# Autodesk Inventor assembly: Hand_tyokudou
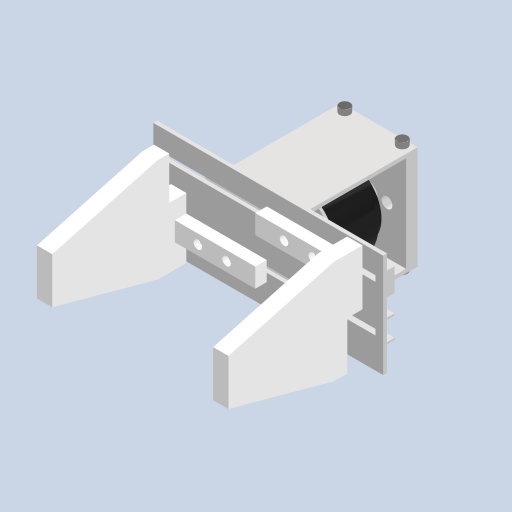
[picture p0: Inventor's stored thumbnail of the model, 512x512]
Saved by Autodesk Inventor 2023 (Build 270158000, 158)
## iProperties
Created: 2024-11-27
Part Number: Hand_tyokudou
Document SubType Name: Assembly
Designer: kiyo
Mass: 142.009 g
Surface Area: 718.919 cm^2
Volume: 132.865 cm^3
Density: 1.06882 g/cm^3
Author: kiyo
## Documents named in this file (14)
- D:\GitHub\inventor\syu-si\OfficeRobot\Manipulator\Hand_tyokudou.iam
- D:\GitHub\inventor\syu-si\OfficeRobot\ReadyMade\Steadywin\GIM3505-8_with-driver.ipt
- D:\GitHub\inventor\syu-si\OfficeRobot\Manipulator\rackgear.ipt
- D:\GitHub\inventor\syu-si\OfficeRobot\Manipulator\motor-fixing.ipt
- D:\GitHub\inventor\syu-si\OfficeRobot\Manipulator\hand-box.ipt
- D:\GitHub\inventor\syu-si\OfficeRobot\Manipulator\left-nail.ipt
- D:\GitHub\inventor\syu-si\OfficeRobot\Manipulator\right-nail.ipt
- D:\GitHub\inventor\syu-si\OfficeRobot\Manipulator\hand-gear.ipt
- D:\GitHub\inventor\syu-si\OfficeRobot\ReadyMade\Screw\GFM-0304-03.ipt
- D:\GitHub\inventor\syu-si\OfficeRobot\ReadyMade\Screw\FB-305530.ipt
- D:\GitHub\inventor\syu-si\OfficeRobot\ReadyMade\Screw\CBSH3-8.ipt
- D:\GitHub\inventor\syu-si\OfficeRobot\Manipulator\connect-wrist.ipt
- D:\GitHub\inventor\syu-si\OfficeRobot\ReadyMade\Screw\M3_6mm.ipt
- D:\GitHub\inventor\syu-si\OfficeRobot\ReadyMade\Screw\M2-5_6mm.ipt
## Components (36 placed, 13 different names)
1. GIM3505-8_with-driver:1 — 挿入:2, 挿入:3
2. left-nail:1 — 挿入:10, 挿入:11, 挿入:20, 挿入:21, フラッシュ:2
3. right-nail:1 — 挿入:14, 挿入:15, 挿入:18, 挿入:19, フラッシュ:1
4. hand-box:1 — メイト:8, メイト:9, 挿入:34, 挿入:35, フラッシュ:1, フラッシュ:2, 挿入:36, 挿入:37, 挿入:38, 挿入:39, 挿入:40, 挿入:41
5. rackgear:1 — 挿入:16, 挿入:17, 挿入:24, 挿入:25
6. rackgear:2 — 挿入:12, 挿入:13, 挿入:22, 挿入:23
7. connect-wrist:1 — 挿入:30, 挿入:31, 挿入:32, 挿入:33, 挿入:34
8. hand-gear — 挿入:42, 挿入:43, 挿入:44
9. motor-fixing:1 — 挿入:2, 挿入:3, 挿入:26, 挿入:27
10. M3_6mm:1 — 挿入:38
11. M3_6mm:2 — 挿入:39
12. M3_6mm:3 — 挿入:40
13. M3_6mm:4 — 挿入:41
14. M3_6mm:5 — 挿入:37
15. M3_6mm:6 — 挿入:36
16. M2-5_6mm:1 — 挿入:44
17. M2-5_6mm:2 — 挿入:43
18. M2-5_6mm:3 — 挿入:42
19. GFM-0304-03:1 — 挿入:10, 挿入:13, メイト:8
20. GFM-0304-03:2 — 挿入:11, 挿入:12
21. GFM-0304-03:3 — 挿入:14, メイト:9, 挿入:16
22. GFM-0304-03:4 — 挿入:15, 挿入:17
23. FB-305530:1 — 挿入:18
24. FB-305530:2 — 挿入:19
25. FB-305530:3 — 挿入:21
26. FB-305530:4 — 挿入:20
27. CBSH3-8:1 — 挿入:25
28. CBSH3-8:2 — 挿入:24
29. CBSH3-8:3 — 挿入:23
30. CBSH3-8:4 — 挿入:22
31. FB-305530:5 — 挿入:27
32. FB-305530:6 — 挿入:26
33. FB-305530:7 — 挿入:31
34. FB-305530:8 — 挿入:30, 挿入:35
35. FB-305530:9 — 挿入:33
36. FB-305530:10 — 挿入:32
## Relationships (44: Insert 38, Mate 4, Flush 2)
- [Insert]: GIM3505-8_with-driver:1 ↔ hand-gear
- [Mate] (0.05 mm): hand-box:1 ↔ rackgear:2
- [Mate] (0.05 mm): hand-box:1 ↔ rackgear:1
- 挿入:2 [Insert]: GIM3505-8_with-driver:1 ↔ motor-fixing:1
- 挿入:3 [Insert]: GIM3505-8_with-driver:1 ↔ motor-fixing:1
- [Insert]: hand-box:1 ↔ motor-fixing:1
- [Insert]: hand-box:1 ↔ motor-fixing:1
- 挿入:10 [Insert]: left-nail:1 ↔ GFM-0304-03:1
- 挿入:11 [Insert]: left-nail:1 ↔ GFM-0304-03:2
- 挿入:12 [Insert]: rackgear:2 ↔ GFM-0304-03:2
- 挿入:13 [Insert]: rackgear:2 ↔ GFM-0304-03:1
- メイト:8 [Mate]: hand-box:1 ↔ GFM-0304-03:1
- 挿入:14 [Insert]: right-nail:1 ↔ GFM-0304-03:3
- 挿入:15 [Insert]: right-nail:1 ↔ GFM-0304-03:4
- メイト:9 [Mate]: hand-box:1 ↔ GFM-0304-03:3
- 挿入:16 [Insert]: rackgear:1 ↔ GFM-0304-03:3
- 挿入:17 [Insert]: rackgear:1 ↔ GFM-0304-03:4
- 挿入:18 [Insert]: right-nail:1 ↔ FB-305530:1
- 挿入:19 [Insert]: right-nail:1 ↔ FB-305530:2
- 挿入:20 [Insert]: left-nail:1 ↔ FB-305530:4
- 挿入:21 [Insert]: left-nail:1 ↔ FB-305530:3
- 挿入:22 [Insert]: rackgear:2 ↔ CBSH3-8:4
- 挿入:23 [Insert]: rackgear:2 ↔ CBSH3-8:3
- 挿入:24 [Insert]: rackgear:1 ↔ CBSH3-8:2
- 挿入:25 [Insert]: rackgear:1 ↔ CBSH3-8:1
- 挿入:26 [Insert]: motor-fixing:1 ↔ FB-305530:6
- 挿入:27 [Insert]: motor-fixing:1 ↔ FB-305530:5
- 挿入:30 [Insert]: connect-wrist:1 ↔ FB-305530:8
- 挿入:31 [Insert]: connect-wrist:1 ↔ FB-305530:7
- 挿入:32 [Insert]: connect-wrist:1 ↔ FB-305530:10
- 挿入:33 [Insert]: connect-wrist:1 ↔ FB-305530:9
- 挿入:34 [Insert]: hand-box:1 ↔ connect-wrist:1
- 挿入:35 [Insert]: hand-box:1 ↔ FB-305530:8
- フラッシュ:1 [Flush] (60 mm): right-nail:1 ↔ hand-box:1
- フラッシュ:2 [Flush] (60 mm): left-nail:1 ↔ hand-box:1
- 挿入:36 [Insert]: hand-box:1 ↔ M3_6mm:6
- 挿入:37 [Insert]: hand-box:1 ↔ M3_6mm:5
- 挿入:38 [Insert]: hand-box:1 ↔ M3_6mm:1
- 挿入:39 [Insert]: hand-box:1 ↔ M3_6mm:2
- 挿入:40 [Insert]: hand-box:1 ↔ M3_6mm:3
- 挿入:41 [Insert]: hand-box:1 ↔ M3_6mm:4
- 挿入:42 [Insert]: hand-gear ↔ M2-5_6mm:3
- 挿入:43 [Insert]: hand-gear ↔ M2-5_6mm:2
- 挿入:44 [Insert]: hand-gear ↔ M2-5_6mm:1
